# Autodesk Inventor assembly: 000-belt_liner_v1
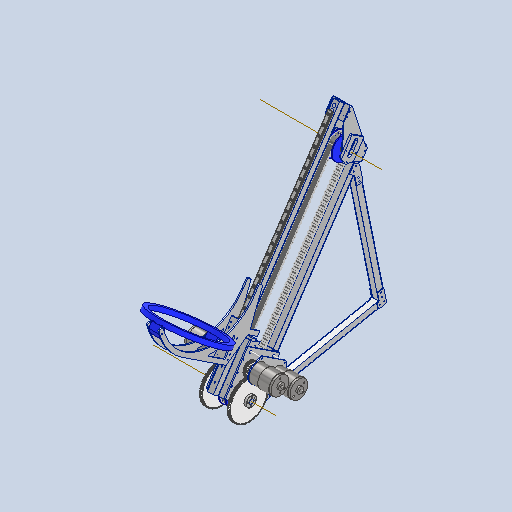
[picture p0: Inventor's stored thumbnail of the model, 512x512]
Saved by Autodesk Inventor 2025.2 (Build 292293000, 293)
## iProperties
Created: 2024-12-08
Part Number: 000-belt_liner_v1
Document SubType Name: Assembly
Designer: haruy
Author: haruy
## Documents named in this file (37)
- C:\Users\haruy\Documents\ロボコン\NHK2025\cad\nagahisa\belt_liner\000-belt_liner_v1.iam
- C:\Users\haruy\Documents\ロボコン\NHK2025\cad\nagahisa\belt_liner\belt_liner_v1_ASP_Base.ipt
- C:\Users\haruy\Documents\ロボコン\NHK2025\cad\nagahisa\belt_liner\SSE2B-MX10-455.iam
- C:\Users\haruy\Documents\ロボコン\NHK2025\cad\nagahisa\belt_liner\belt_liner_v1_Plate_1.ipt
- C:\Users\haruy\Documents\ロボコン\NHK2025\cad\nagahisa\belt_liner\belt_liner_v1_Plate_2.ipt
- C:\Users\haruy\Documents\ロボコン\NHK2025\cad\nagahisa\belt_liner\belt_liner_v1_Plate_3.ipt
- C:\Users\haruy\Documents\ロボコン\NHK2025\cad\000_parts\ベアリング\10\bear_10_15_sn.ipt
- C:\Users\haruy\Documents\ロボコン\NHK2025\cad\nagahisa\belt_liner\belt_liner_v1_shaft_spesa-25.ipt
- C:\Users\haruy\Documents\ロボコン\NHK2025\cad\nagahisa\belt_liner\belt_liner_v1_Plate_4.ipt
- C:\Users\haruy\Documents\ロボコン\NHK2025\cad\nagahisa\belt_liner\belt_liner_v1_Plate_5.ipt
- C:\Users\haruy\Documents\ロボコン\NHK2025\cad\000_parts\エンコーダー\encoder v2.ipt
- C:\Users\haruy\Documents\ロボコン\NHK2025\cad\nagahisa\belt_liner\belt_liner_v1_Plate_6.ipt
- C:\Users\haruy\Documents\ロボコン\NHK2025\cad\nagahisa\belt_liner\belt_liner_v1_Plate_7.ipt
- C:\Users\haruy\Documents\ロボコン\NHK2025\cad\nagahisa\belt_liner\belt_liner_v1_Plate_8.ipt
- C:\Users\haruy\Documents\ロボコン\NHK2025\cad\nagahisa\belt_liner\belt_liner_v1_Plate_9.ipt
- C:\Users\haruy\Documents\ロボコン\NHK2025\cad\nagahisa\belt_liner\000-belt_liner_v1\デザイン アクセラレータ\歯付きベルト伝達1.iam
- C:\Users\haruy\Documents\ロボコン\NHK2025\cad\nagahisa\belt_liner\belt_liner_v1_shaft-54.ipt
- C:\Users\haruy\Documents\ロボコン\NHK2025\cad\nagahisa\belt_liner\SCSWJ10-6.iam
- C:\Users\haruy\Documents\ロボコン\NHK2025\cad\nagahisa\belt_liner\belt_liner_v1_shaft-84.ipt
- C:\Users\haruy\Documents\ロボコン\NHK2025\cad\nagahisa\belt_liner\000-belt_liner_v1\デザイン アクセラレータ\平歯車1.iam
- C:\Users\haruy\Documents\ロボコン\NHK2025\cad\nagahisa\belt_liner\belt_liner_v1_3DP_spesa-1.ipt
- C:\Users\haruy\Documents\ロボコン\NHK2025\cad\nagahisa\belt_liner\belt_liner_v1_3DP_spesa-2.ipt
- C:\Users\haruy\Documents\ロボコン\NHK2025\cad\nagahisa\belt_liner\belt_liner_v1_MDF_throw_plate.ipt
- C:\Users\haruy\Documents\ロボコン\NHK2025\cad\nagahisa\belt_liner\belt_liner_v1_Plate_10.ipt
- C:\Users\haruy\Documents\ロボコン\NHK2025\cad\nagahisa\belt_liner\belt_liner_v1_Plate_11.ipt
- C:\Users\haruy\Documents\ロボコン\NHK2025\cad\nagahisa\belt_liner\belt_liner_v1_Plate_12.ipt
- C:\Users\haruy\Documents\ロボコン\NHK2025\cad\nagahisa\belt_liner\belt_liner_v1_Plate_13.ipt
- C:\Users\haruy\Documents\ロボコン\NHK2025\cad\nagahisa\belt_liner\belt_liner_v1_Plate_14.ipt
- C:\Users\haruy\Documents\ロボコン\NHK2025\cad\nagahisa\belt_liner\belt_liner_v1_Plate_15.ipt
- C:\Users\haruy\Documents\ロボコン\NHK2025\cad\nagahisa\belt_liner\000-belt_liner_v1\デザイン アクセラレータ\平歯車2.iam
- C:\Users\haruy\Documents\ロボコン\NHK2025\cad\nagahisa\dribl\R2-Rzvector\RZvector-v1-3DP-E-F.ipt
- C:\Users\haruy\Documents\ロボコン\NHK2025\cad\nagahisa\belt_liner\rs735.ipt
- C:\Users\haruy\Documents\ロボコン\NHK2025\cad\nagahisa\belt_liner\setcorer_5-10-22.ipt
- C:\Users\haruy\Documents\ロボコン\NHK2025\cad\nagahisa\belt_liner\000-belt_liner_v1\デザイン アクセラレータ\平歯車3.iam
- C:\Users\haruy\Documents\ロボコン\NHK2025\cad\nagahisa\belt_liner\belt_liner_v1_3DP_P_F-1.ipt
- C:\Users\haruy\Documents\ロボコン\NHK2025\cad\nagahisa\belt_liner\belt_liner_v1_3DP_P_F-2.ipt
- C:\Users\haruy\Documents\ロボコン\NHK2025\cad\nagahisa\belt_liner\belt_liner_v1_3DP_C_ring.ipt
## Components (60 placed, 34 different names)
1. belt_liner_v1_ASP_Base:1 — 挿入:1, 挿入:2, 挿入:3, 挿入:4, 挿入:5, 挿入:6, フラッシュ:1, 挿入:62, 挿入:63, 挿入:64, 挿入:65, 挿入:66, 挿入:67, 挿入:68, 挿入:69, 挿入:70, 挿入:71, 挿入:72, 挿入:73, 挿入:124, 挿入:125, 挿入:145, 挿入:146
2. SSE2B-MX10-455:1 [sub-assembly] — 挿入:1, 挿入:2, 挿入:134, 挿入:135
3. belt_liner_v1_Plate_1:1 — 挿入:3, 挿入:4
4. belt_liner_v1_Plate_2:1 — 挿入:5, 挿入:6, 挿入:7, 挿入:10, 挿入:103
5. belt_liner_v1_Plate_3:1 — 挿入:7, 挿入:12, 挿入:89, 挿入:90, 挿入:91, 挿入:103
6. belt_liner_v1_Plate_3:2 — 挿入:10, 挿入:11, 挿入:94, 挿入:95, 挿入:96
7. bear_10_15_sn:1 — 挿入:11, 挿入:55
8. bear_10_15_sn:2 — 挿入:12, 挿入:50
9. encoder v2:1 — 挿入:99, 挿入:100
10. belt_liner_v1_Plate_6:1 — 挿入:124, 挿入:125, 挿入:127, 挿入:128, 挿入:130
11. belt_liner_v1_Plate_7:1 — 挿入:143, 挿入:144, 挿入:145, 挿入:146
12. belt_liner_v1_Plate_8:1 — 挿入:121, 挿入:122, 挿入:127, 挿入:128, 挿入:143, 挿入:144
13. belt_liner_v1_Plate_8:2 — 挿入:130, 挿入:131, 挿入:132
14. belt_liner_v1_Plate_9:1 — 挿入:131, 挿入:132
15. belt_liner_v1_Plate_9:2 — 正接:1, 挿入:121, 挿入:122
16. 歯付きベルト伝達:1 [sub-assembly] — 挿入:41, 挿入:49, メイト:5, メイト:6, 挿入:109, 挿入:126, 挿入:133
17. bear_10_15_sn:3 — 挿入:42, 挿入:47, 挿入:123
18. bear_10_15_sn:4 — 挿入:41, 挿入:48
19. belt_liner_v1_shaft-54:1 — 挿入:42, 正接:1
20. SCSWJ10-6:1 [sub-assembly] — 挿入:44, 挿入:104, 挿入:110
21. belt_liner_v1_shaft-84:1 — 挿入:44, 挿入:45, 挿入:46, メイト:7
22. SCSWJ10-6:2 [sub-assembly] — 挿入:45
23. SCSWJ10-6:3 [sub-assembly] — 挿入:46
24. 平歯車:1 [sub-assembly] — メイト:7, メイト:8, メイト:9
25. belt_liner_v1_3DP_spesa-1:1 — 挿入:47
26. belt_liner_v1_3DP_spesa-1:2 — 挿入:48
27. belt_liner_v1_3DP_spesa-1:3 — 挿入:49, 挿入:55
28. belt_liner_v1_3DP_spesa-2:1 — 挿入:50, 挿入:104
29. belt_liner_v1_MDF_throw_plate:1 — 挿入:134, 挿入:135, 挿入:136, 挿入:137, 挿入:138, 挿入:139
30. belt_liner_v1_Plate_10:1 — 挿入:136, 挿入:137, 挿入:140
31. belt_liner_v1_Plate_11:1 — 挿入:64, 挿入:65
32. belt_liner_v1_Plate_11:2 — 挿入:62, 挿入:63
33. belt_liner_v1_Plate_12:1 — 挿入:68, 挿入:69
34. belt_liner_v1_Plate_12:2 — 挿入:66, 挿入:67
35. belt_liner_v1_Plate_13:1 — 挿入:72, 挿入:73
36. belt_liner_v1_Plate_13:2 — 挿入:70, 挿入:71
37. belt_liner_v1_Plate_14:1 — 挿入:84, 挿入:85
38. belt_liner_v1_Plate_15:1 — 挿入:84, 挿入:85, メイト:5, メイト:6
39. 平歯車:2 [sub-assembly] — 挿入:87, 挿入:88, 挿入:100
40. RZvector-v1-3DP-E-F:1 — 挿入:87, 挿入:88
41. belt_liner_v1_shaft_spesa-25:1 — 挿入:91, 挿入:92
42. belt_liner_v1_shaft_spesa-25:3 — 挿入:89
43. belt_liner_v1_shaft_spesa-25:4 — 挿入:90, 挿入:93
44. belt_liner_v1_Plate_4:1 — 挿入:92, 挿入:93, 挿入:105, 挿入:106
45. belt_liner_v1_Plate_5:1 — 挿入:97, 挿入:98, 挿入:99, 挿入:101
46. belt_liner_v1_shaft_spesa-25:5 — 挿入:94, 挿入:98
47. belt_liner_v1_shaft_spesa-25:6 — 挿入:95
48. belt_liner_v1_shaft_spesa-25:7 — 挿入:96, 挿入:97
49. rs735:1 — 挿入:101, 挿入:102, メイト:9
50. setcorer_5-10-22:1 — 挿入:102, メイト:8
51. rs735:2 — 挿入:105, 挿入:107
52. rs735:3 — 挿入:106, 挿入:108, メイト:10
53. 平歯車:3 [sub-assembly]
54. setcorer_5-10-22:2 — 挿入:107
55. setcorer_5-10-22:3 — 挿入:108, メイト:11
56. 平歯車:4 [sub-assembly] — メイト:10, メイト:11
57. belt_liner_v1_3DP_P_F-1:1 — 挿入:109, 挿入:110
58. belt_liner_v1_3DP_P_F-2:1 — 挿入:123, 挿入:126, 挿入:133
59. belt_liner_v1_Plate_10:2 — 挿入:138, 挿入:139, 挿入:141, 挿入:142
60. belt_liner_v1_3DP_C_ring:1 — 挿入:140, 挿入:141, 挿入:142
## Relationships (92: Insert 83, Mate 7, Flush 1, Tangent 1)
- 挿入:1 [Insert]: belt_liner_v1_ASP_Base:1 ↔ SSE2B-MX10-455:1
- 挿入:2 [Insert]: belt_liner_v1_ASP_Base:1 ↔ SSE2B-MX10-455:1
- 挿入:3 [Insert]: belt_liner_v1_ASP_Base:1 ↔ belt_liner_v1_Plate_1:1
- 挿入:4 [Insert]: belt_liner_v1_ASP_Base:1 ↔ belt_liner_v1_Plate_1:1
- 挿入:5 [Insert]: belt_liner_v1_ASP_Base:1 ↔ belt_liner_v1_Plate_2:1
- 挿入:6 [Insert]: belt_liner_v1_ASP_Base:1 ↔ belt_liner_v1_Plate_2:1
- 挿入:7 [Insert]: belt_liner_v1_Plate_2:1 ↔ belt_liner_v1_Plate_3:1
- 挿入:10 [Insert]: belt_liner_v1_Plate_2:1 ↔ belt_liner_v1_Plate_3:2
- 挿入:11 [Insert]: belt_liner_v1_Plate_3:2 ↔ bear_10_15_sn:1
- 挿入:12 [Insert]: belt_liner_v1_Plate_3:1 ↔ bear_10_15_sn:2
- フラッシュ:1 [Flush] (-7.5 mm): belt_liner_v1_ASP_Base:1
- 挿入:41 [Insert]: 歯付きベルト伝達:1 ↔ bear_10_15_sn:4
- 挿入:42 [Insert] (-16.5 mm): bear_10_15_sn:3 ↔ belt_liner_v1_shaft-54:1
- 挿入:44 [Insert] (-26.5 mm): SCSWJ10-6:1 ↔ belt_liner_v1_shaft-84:1
- 挿入:45 [Insert]: belt_liner_v1_shaft-84:1 ↔ SCSWJ10-6:2
- 挿入:46 [Insert]: belt_liner_v1_shaft-84:1 ↔ SCSWJ10-6:3
- 挿入:47 [Insert]: bear_10_15_sn:3 ↔ belt_liner_v1_3DP_spesa-1:1
- 挿入:48 [Insert]: bear_10_15_sn:4 ↔ belt_liner_v1_3DP_spesa-1:2
- 挿入:49 [Insert]: 歯付きベルト伝達:1 ↔ belt_liner_v1_3DP_spesa-1:3
- 挿入:50 [Insert]: bear_10_15_sn:2 ↔ belt_liner_v1_3DP_spesa-2:1
- 挿入:55 [Insert]: bear_10_15_sn:1 ↔ belt_liner_v1_3DP_spesa-1:3
- 正接:1 [Tangent]: belt_liner_v1_Plate_9:2 ↔ belt_liner_v1_shaft-54:1
- 挿入:62 [Insert]: belt_liner_v1_ASP_Base:1 ↔ belt_liner_v1_Plate_11:2
- 挿入:63 [Insert]: belt_liner_v1_ASP_Base:1 ↔ belt_liner_v1_Plate_11:2
- 挿入:64 [Insert]: belt_liner_v1_ASP_Base:1 ↔ belt_liner_v1_Plate_11:1
- 挿入:65 [Insert]: belt_liner_v1_ASP_Base:1 ↔ belt_liner_v1_Plate_11:1
- 挿入:66 [Insert]: belt_liner_v1_ASP_Base:1 ↔ belt_liner_v1_Plate_12:2
- 挿入:67 [Insert]: belt_liner_v1_ASP_Base:1 ↔ belt_liner_v1_Plate_12:2
- 挿入:68 [Insert]: belt_liner_v1_ASP_Base:1 ↔ belt_liner_v1_Plate_12:1
- 挿入:69 [Insert]: belt_liner_v1_ASP_Base:1 ↔ belt_liner_v1_Plate_12:1
- 挿入:70 [Insert]: belt_liner_v1_ASP_Base:1 ↔ belt_liner_v1_Plate_13:2
- 挿入:71 [Insert]: belt_liner_v1_ASP_Base:1 ↔ belt_liner_v1_Plate_13:2
- 挿入:72 [Insert]: belt_liner_v1_ASP_Base:1 ↔ belt_liner_v1_Plate_13:1
- 挿入:73 [Insert]: belt_liner_v1_ASP_Base:1 ↔ belt_liner_v1_Plate_13:1
- 挿入:84 [Insert]: belt_liner_v1_Plate_14:1 ↔ belt_liner_v1_Plate_15:1
- 挿入:85 [Insert]: belt_liner_v1_Plate_14:1 ↔ belt_liner_v1_Plate_15:1
- メイト:5 [Mate]: 歯付きベルト伝達:1 ↔ belt_liner_v1_Plate_15:1
- メイト:6 [Mate]: 歯付きベルト伝達:1 ↔ belt_liner_v1_Plate_15:1
- 挿入:87 [Insert]: 平歯車:2 ↔ RZvector-v1-3DP-E-F:1
- 挿入:88 [Insert]: 平歯車:2 ↔ RZvector-v1-3DP-E-F:1
- 挿入:89 [Insert]: belt_liner_v1_Plate_3:1 ↔ belt_liner_v1_shaft_spesa-25:3
- 挿入:90 [Insert]: belt_liner_v1_Plate_3:1 ↔ belt_liner_v1_shaft_spesa-25:4
- 挿入:91 [Insert]: belt_liner_v1_Plate_3:1 ↔ belt_liner_v1_shaft_spesa-25:1
- 挿入:92 [Insert]: belt_liner_v1_shaft_spesa-25:1 ↔ belt_liner_v1_Plate_4:1
- 挿入:93 [Insert]: belt_liner_v1_shaft_spesa-25:4 ↔ belt_liner_v1_Plate_4:1
- 挿入:94 [Insert]: belt_liner_v1_Plate_3:2 ↔ belt_liner_v1_shaft_spesa-25:5
- 挿入:95 [Insert]: belt_liner_v1_Plate_3:2 ↔ belt_liner_v1_shaft_spesa-25:6
- 挿入:96 [Insert]: belt_liner_v1_Plate_3:2 ↔ belt_liner_v1_shaft_spesa-25:7
- 挿入:97 [Insert]: belt_liner_v1_Plate_5:1 ↔ belt_liner_v1_shaft_spesa-25:7
- 挿入:98 [Insert]: belt_liner_v1_Plate_5:1 ↔ belt_liner_v1_shaft_spesa-25:5
- 挿入:99 [Insert]: encoder v2:1 ↔ belt_liner_v1_Plate_5:1
- 挿入:100 [Insert] (2 mm): encoder v2:1 ↔ 平歯車:2
- 挿入:101 [Insert]: belt_liner_v1_Plate_5:1 ↔ rs735:1
- 挿入:102 [Insert]: rs735:1 ↔ setcorer_5-10-22:1
- メイト:7 [Mate]: belt_liner_v1_shaft-84:1 ↔ 平歯車:1
- メイト:8 [Mate]: 平歯車:1 ↔ setcorer_5-10-22:1
- メイト:9 [Mate]: 平歯車:1 ↔ rs735:1
- 挿入:103 [Insert]: belt_liner_v1_Plate_2:1 ↔ belt_liner_v1_Plate_3:1
- 挿入:104 [Insert]: SCSWJ10-6:1 ↔ belt_liner_v1_3DP_spesa-2:1
- 挿入:105 [Insert]: belt_liner_v1_Plate_4:1 ↔ rs735:2
- 挿入:106 [Insert]: belt_liner_v1_Plate_4:1 ↔ rs735:3
- 挿入:107 [Insert]: rs735:2 ↔ setcorer_5-10-22:2
- 挿入:108 [Insert]: rs735:3 ↔ setcorer_5-10-22:3
- メイト:10 [Mate]: rs735:3 ↔ 平歯車:4
- メイト:11 [Mate]: setcorer_5-10-22:3 ↔ 平歯車:4
- 挿入:109 [Insert]: 歯付きベルト伝達:1 ↔ belt_liner_v1_3DP_P_F-1:1
- 挿入:110 [Insert]: SCSWJ10-6:1 ↔ belt_liner_v1_3DP_P_F-1:1
- 挿入:121 [Insert]: belt_liner_v1_Plate_8:1 ↔ belt_liner_v1_Plate_9:2
- 挿入:122 [Insert]: belt_liner_v1_Plate_8:1 ↔ belt_liner_v1_Plate_9:2
- 挿入:123 [Insert]: bear_10_15_sn:3 ↔ belt_liner_v1_3DP_P_F-2:1
- 挿入:124 [Insert]: belt_liner_v1_ASP_Base:1 ↔ belt_liner_v1_Plate_6:1
- 挿入:125 [Insert]: belt_liner_v1_ASP_Base:1 ↔ belt_liner_v1_Plate_6:1
- 挿入:126 [Insert]: 歯付きベルト伝達:1 ↔ belt_liner_v1_3DP_P_F-2:1
- 挿入:127 [Insert]: belt_liner_v1_Plate_6:1 ↔ belt_liner_v1_Plate_8:1
- 挿入:128 [Insert]: belt_liner_v1_Plate_6:1 ↔ belt_liner_v1_Plate_8:1
- 挿入:130 [Insert]: belt_liner_v1_Plate_6:1 ↔ belt_liner_v1_Plate_8:2
- 挿入:131 [Insert]: belt_liner_v1_Plate_8:2 ↔ belt_liner_v1_Plate_9:1
- 挿入:132 [Insert]: belt_liner_v1_Plate_8:2 ↔ belt_liner_v1_Plate_9:1
- 挿入:133 [Insert]: 歯付きベルト伝達:1 ↔ belt_liner_v1_3DP_P_F-2:1
- 挿入:134 [Insert]: SSE2B-MX10-455:1 ↔ belt_liner_v1_MDF_throw_plate:1
- 挿入:135 [Insert]: SSE2B-MX10-455:1 ↔ belt_liner_v1_MDF_throw_plate:1
- 挿入:136 [Insert]: belt_liner_v1_MDF_throw_plate:1 ↔ belt_liner_v1_Plate_10:1
- 挿入:137 [Insert]: belt_liner_v1_MDF_throw_plate:1 ↔ belt_liner_v1_Plate_10:1
- 挿入:138 [Insert]: belt_liner_v1_MDF_throw_plate:1 ↔ belt_liner_v1_Plate_10:2
- 挿入:139 [Insert]: belt_liner_v1_MDF_throw_plate:1 ↔ belt_liner_v1_Plate_10:2
- 挿入:140 [Insert]: belt_liner_v1_Plate_10:1 ↔ belt_liner_v1_3DP_C_ring:1
- 挿入:141 [Insert]: belt_liner_v1_Plate_10:2 ↔ belt_liner_v1_3DP_C_ring:1
- 挿入:142 [Insert]: belt_liner_v1_Plate_10:2 ↔ belt_liner_v1_3DP_C_ring:1
- 挿入:143 [Insert]: belt_liner_v1_Plate_7:1 ↔ belt_liner_v1_Plate_8:1
- 挿入:144 [Insert]: belt_liner_v1_Plate_7:1 ↔ belt_liner_v1_Plate_8:1
- 挿入:145 [Insert]: belt_liner_v1_ASP_Base:1 ↔ belt_liner_v1_Plate_7:1
- 挿入:146 [Insert]: belt_liner_v1_ASP_Base:1 ↔ belt_liner_v1_Plate_7:1
